# Autodesk Inventor assembly: RC Car
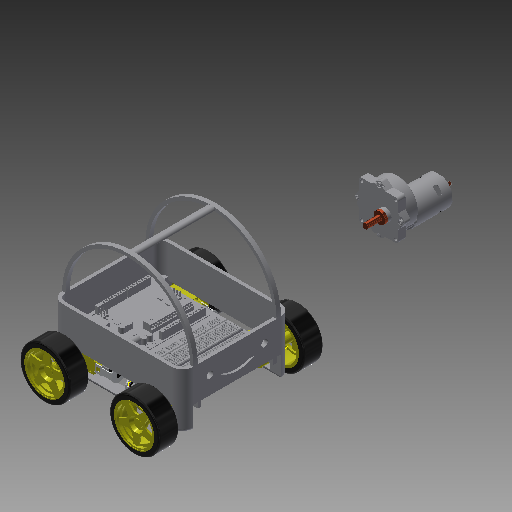
[picture p0: Inventor's stored thumbnail of the model, 512x512]
Saved by Autodesk Inventor 2019 (Build 230136000, 136)
## iProperties
Created: 2020-12-04
Part Number: RC Car
Document SubType Name: Assembly
Designer: melis
Author: melis
## Documents named in this file (7)
- C:\Users\melis\OneDrive\Desktop\Code&Mech\InventorParts\RC Car.iam
- C:\Users\melis\OneDrive\Desktop\Code&Mech\InventorParts\rc car inards\breadboard_350_pos_asm.ipt
- C:\Users\melis\OneDrive\Desktop\Code&Mech\InventorParts\rc car inards\Arduino Uno.ipt
- C:\Users\melis\Downloads\dc-gear-motor-1.snapshot.1\Model 302 DC Gearmotor.ipt
- C:\Users\melis\OneDrive\Desktop\Code&Mech\InventorParts\rc car inards\motor.ipt
- C:\Users\melis\OneDrive\Desktop\Code&Mech\InventorParts\chassis.ipt
- C:\Users\melis\OneDrive\Desktop\Code&Mech\InventorParts\rc car inards\velg.ipt
## Components (12 placed, 6 different names)
1. breadboard_350_pos_asm:1 — Mate:6
2. Arduino Uno:1 — Tangent:1, Mate:5
3. Model 302 DC Gearmotor:3 — Tangent:1
4. motor:1 — Mate:7, Mate:8, Rigid:4, Mate:14
5. motor:2 — Mate:3, Mate:4, Rigid:2, Mate:13
6. motor:3 — Mate:1, Mate:2, Rigid:1, Mate:11, Mate:12
7. motor:4 — Mate:9, Mate:10, Rigid:3, Mate:15
8. chassis:1 — Mate:1, Mate:2, Mate:3, Mate:4, Mate:5, Mate:6, Mate:7, Mate:8, Mate:9, Mate:10, Mate:11, Mate:12, Mate:13, Mate:14, Mate:15
9. velg:1 — Rigid:2
10. velg:2 — Rigid:3
11. velg:3 — Rigid:4
12. velg:4 — Rigid:1
## Relationships (20: Mate 15, WeldJoint 4, Tangent 1)
- Tangent:1: Arduino Uno:1 ↔ Model 302 DC Gearmotor:3
- Mate:1: motor:3 ↔ chassis:1
- Mate:2: motor:3 ↔ chassis:1
- Mate:3: motor:2 ↔ chassis:1
- Mate:4: motor:2 ↔ chassis:1
- Rigid:1 [WeldJoint]: motor:3 ↔ velg:4
- Rigid:2 [WeldJoint]: motor:2 ↔ velg:1
- Mate:5: Arduino Uno:1 ↔ chassis:1
- Mate:6: breadboard_350_pos_asm:1 ↔ chassis:1
- Mate:7: motor:1 ↔ chassis:1
- Mate:8: motor:1 ↔ chassis:1
- Mate:9: motor:4 ↔ chassis:1
- Mate:10: motor:4 ↔ chassis:1
- Rigid:3 [WeldJoint]: motor:4 ↔ velg:2
- Rigid:4 [WeldJoint]: motor:1 ↔ velg:3
- Mate:11: motor:3 ↔ chassis:1
- Mate:12: motor:3 ↔ chassis:1
- Mate:13: motor:2 ↔ chassis:1
- Mate:14: motor:1 ↔ chassis:1
- Mate:15: motor:4 ↔ chassis:1
